# Autodesk Inventor assembly: ASY SLM 0100 frame
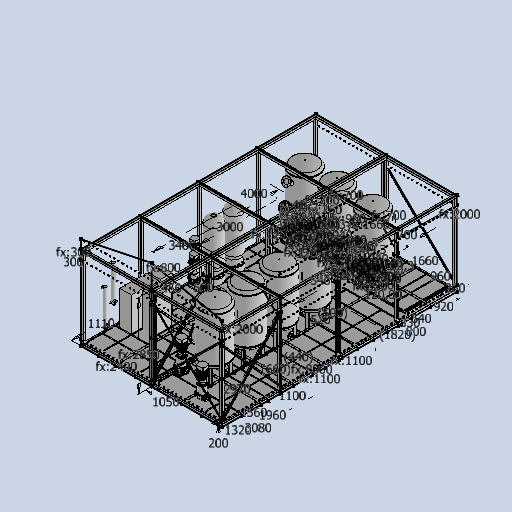
[picture p0: Inventor's stored thumbnail of the model, 512x512]
Saved by Autodesk Inventor 2025.3 (Build 293356030, 356C)
## iProperties
Created: 2025-12-15
Part Number: ASY SLM 0100 frame
Document SubType Name: Assembly
Designer: admin
Author: admin
## Documents named in this file (11)
- C:\Users\admin\Yandex.Disk\home pc\Inventor\SLM-Salemal\ASY SLM 0100 frame.iam
- C:\Users\admin\Yandex.Disk\home pc\Inventor\SLM-Salemal\ASY SLM 1600 Filter column D1000.iam
- C:\Users\admin\Yandex.Disk\home pc\Inventor\SLM-Salemal\Оборудование Инвентор\HY-H H2162–4T.ipt
- C:\Users\admin\Yandex.Disk\home pc\Inventor\SLM-Salemal\Оборудование Инвентор\UV-Cleaner ODV-15.ipt
- C:\Users\admin\Yandex.Disk\home pc\Inventor\SLM-Salemal\Оборудование Инвентор\Станции дозирования\Coagulant barrel.ipt
- C:\Users\admin\Yandex.Disk\home pc\Inventor\SLM-Salemal\Оборудование Инвентор\Станции дозирования\Flocculant barrel.ipt
- C:\Users\admin\Yandex.Disk\home pc\Inventor\SLM-Salemal\Оборудование Инвентор\Станции дозирования\GPHN barrel.ipt
- C:\Users\admin\Yandex.Disk\home pc\Inventor\SLM-Salemal\Оборудование Инвентор\Станции дозирования\Soda barrel.ipt
- C:\Users\admin\Yandex.Disk\home pc\Inventor\SLM-Salemal\Оборудование Инвентор\Вертикальный насос\CDM(F)15-4 FSWP(S_L)C\CDM(F)15-4 FSWP(S_L)C.iam
- C:\Users\admin\Yandex.Disk\home pc\Inventor\SLM-Salemal\Оборудование Инвентор\Вертикальный насос\CDM(F)65-2-2 FSWP(S)C\CDM(F)65-2-2 FSWP(S)C.iam
- C:\Users\admin\Yandex.Disk\home pc\Inventor\SLM-Salemal\ASY SLM 1110 MAIN FRAME.iam
## Components (21 placed, 10 different names)
1. HY-H H2162–4T:1 — Mate:16
2. UV-Cleaner ODV-15:1
3. Coagulant barrel:1
4. Flocculant barrel:1
5. GPHN barrel:1
6. Soda barrel:1
7. CDM(F)65-2-2 FSWP(S)C:1 [sub-assembly]
8. HY-H H2162–4T:2 — Mate:15
9. CDM(F)15-4 FSWP(S_L)C:2 [sub-assembly]
10. CDM(F)65-2-2 FSWP(S)C:2 [sub-assembly]
11. UV-Cleaner ODV-15:2
12. ASY SLM 1110 MAIN FRAME:1 [sub-assembly] — Flush:1, Mate:12, Mate:13, Mate:15, Mate:16
13. ASY SLM 1600 Filter column D1000:16 [sub-assembly]
14. CDM(F)15-4 FSWP(S_L)C:5 [sub-assembly]
15. ASY SLM 1600 Filter column D1000:24 [sub-assembly] — Flush:1, Mate:12, Flush:2, Mate:13, Flush:3, Flush:4, Flush:5, Flush:6, Flush:7, Flush:8, Flush:9, Flush:10, Flush:11
16. ASY SLM 1600 Filter column D1000:20 [sub-assembly] — Flush:2, Flush:3, Flush:11, Flush:12
17. ASY SLM 1600 Filter column D1000:26 [sub-assembly] — Flush:4, Flush:9, Flush:12, Flush:13
18. ASY SLM 1600 Filter column D1000:23 [sub-assembly] — Flush:5, Flush:10, Flush:13
19. ASY SLM 1600 Filter column D1000:7 [sub-assembly] — Flush:8
20. ASY SLM 1600 Filter column D1000:22 [sub-assembly] — Flush:6
21. ASY SLM 1600 Filter column D1000:25 [sub-assembly] — Flush:7
## Relationships (18: Flush 13, Mate 5)
- [Mate]: ASY SLM 1110 MAIN FRAME:1
- Flush:1 (300 mm): ASY SLM 1110 MAIN FRAME:1 ↔ ASY SLM 1600 Filter column D1000:24
- Mate:12: ASY SLM 1110 MAIN FRAME:1 ↔ ASY SLM 1600 Filter column D1000:24
- Flush:2: ASY SLM 1600 Filter column D1000:24 ↔ ASY SLM 1600 Filter column D1000:20
- Mate:13 (-1310 mm): ASY SLM 1110 MAIN FRAME:1 ↔ ASY SLM 1600 Filter column D1000:24
- Flush:3: ASY SLM 1600 Filter column D1000:24 ↔ ASY SLM 1600 Filter column D1000:20
- Flush:4: ASY SLM 1600 Filter column D1000:24 ↔ ASY SLM 1600 Filter column D1000:26
- Flush:5: ASY SLM 1600 Filter column D1000:24 ↔ ASY SLM 1600 Filter column D1000:23
- Flush:6: ASY SLM 1600 Filter column D1000:24 ↔ ASY SLM 1600 Filter column D1000:22
- Flush:7: ASY SLM 1600 Filter column D1000:24 ↔ ASY SLM 1600 Filter column D1000:25
- Flush:8: ASY SLM 1600 Filter column D1000:24 ↔ ASY SLM 1600 Filter column D1000:7
- Flush:9: ASY SLM 1600 Filter column D1000:24 ↔ ASY SLM 1600 Filter column D1000:26
- Flush:10: ASY SLM 1600 Filter column D1000:24 ↔ ASY SLM 1600 Filter column D1000:23
- Flush:11 (-1100 mm): ASY SLM 1600 Filter column D1000:24 ↔ ASY SLM 1600 Filter column D1000:20
- Flush:12 (-1100 mm): ASY SLM 1600 Filter column D1000:20 ↔ ASY SLM 1600 Filter column D1000:26
- Flush:13 (1100 mm): ASY SLM 1600 Filter column D1000:26 ↔ ASY SLM 1600 Filter column D1000:23
- Mate:15: HY-H H2162–4T:2 ↔ ASY SLM 1110 MAIN FRAME:1
- Mate:16: HY-H H2162–4T:1 ↔ ASY SLM 1110 MAIN FRAME:1
